# Autodesk Inventor assembly: Lock Collar Assembly (plastic)
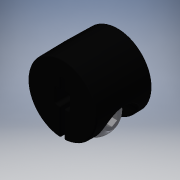
[picture p0: Inventor's stored thumbnail of the model, 180x180]
Saved by Autodesk Inventor 2017 SP1 (Build 210196100, 196)
## iProperties
Created: 2016-12-21
Part Number: Lock Collar Assembly (plastic)
Document SubType Name: Assembly
Designer: brand
Author: brand
## Documents named in this file (4)
- D:\brand\Documents\GrabCAD\SIGBots CAD Library\Motion\Lock Collar Assembly (plastic).iam
- D:\brand\Documents\GrabCAD\SIGBots CAD Library\Motion\Lock Collar (plastic).ipt
- D:\brand\Documents\GrabCAD\SIGBots CAD Library\Structure\Lock Nut.ipt
- D:\brand\Documents\GrabCAD\SIGBots CAD Library\Structure\Bolt 0.375 inch.ipt
## Components (3 placed, 3 different names)
1. Lock Collar (plastic):1 — Mate:6, Mate:8
2. Lock Nut:1 — Mate:7, Mate:8
3. Bolt 0.375 inch:1 — Mate:6, Mate:7
## Relationships (3: Mate 3)
- Mate:6: Lock Collar (plastic):1 ↔ Bolt 0.375 inch:1
- Mate:7: Lock Nut:1 ↔ Bolt 0.375 inch:1
- Mate:8: Lock Collar (plastic):1 ↔ Lock Nut:1
